# Autodesk Inventor assembly: tiller assembly
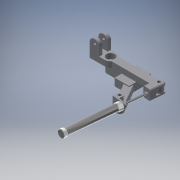
[picture p0: Inventor's stored thumbnail of the model, 180x180]
Saved by Autodesk Inventor 2017 (Build 210142000, 142)
## iProperties
Created: 2017-12-08
Part Number: tiller assembly
Document SubType Name: Assembly
Designer: RLanting
Author: RLanting
## Documents named in this file (6)
- E:\direct drive electronic valving 2\hydraulic steering\tiller assembly.iam
- E:\direct drive electronic valving 2\hydraulic steering\CJ2B16-100Z.iam
- E:\direct drive electronic valving 2\hydraulic steering\tiller frame bracket.ipt
- E:\direct drive electronic valving 2\hydraulic steering\tiller rotation bracket.ipt
- E:\direct drive electronic valving 2\hydraulic steering\cylinder clevis.ipt
- E:\direct drive electronic valving 2\hydraulic steering\cylinder bracket.ipt
## Components (5 placed, 5 different names)
1. CJ2B16-100Z:1 [sub-assembly] — Mate:3, Mate:4, Mate:7, Mate:8
2. tiller frame bracket:1 — Mate:1, Mate:2, Angle:1, Mate:9, Angle:2
3. tiller rotation bracket:1 — Mate:1, Mate:2, Mate:5, Mate:6, Angle:2
4. cylinder clevis:1 — Mate:3, Mate:4, Mate:5, Mate:6
5. cylinder bracket:1 — Mate:7, Mate:8, Angle:1, Mate:9
## Relationships (11: Mate 9, Angle 2)
- Mate:1: tiller frame bracket:1 ↔ tiller rotation bracket:1
- Mate:2: tiller frame bracket:1 ↔ tiller rotation bracket:1
- Mate:3: CJ2B16-100Z:1 ↔ cylinder clevis:1
- Mate:4: CJ2B16-100Z:1 ↔ cylinder clevis:1
- Mate:5: tiller rotation bracket:1 ↔ cylinder clevis:1
- Mate:6: tiller rotation bracket:1 ↔ cylinder clevis:1
- Mate:7: CJ2B16-100Z:1 ↔ cylinder bracket:1
- Mate:8: CJ2B16-100Z:1 ↔ cylinder bracket:1
- Angle:1 (0 deg): tiller frame bracket:1 ↔ cylinder bracket:1
- Mate:9: tiller frame bracket:1 ↔ cylinder bracket:1
- Angle:2 (0 deg): tiller frame bracket:1 ↔ tiller rotation bracket:1
